# Autodesk Inventor assembly: base
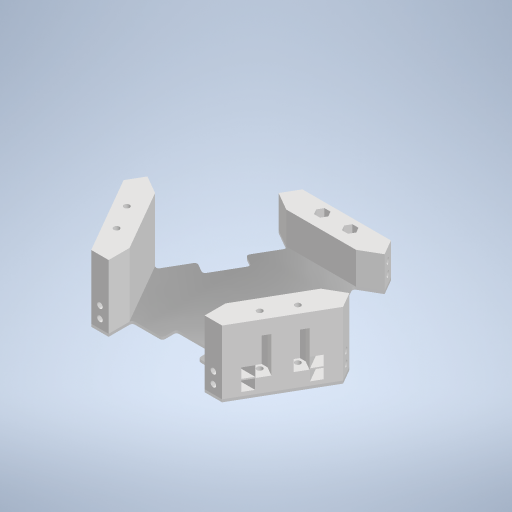
[picture p0: Inventor's stored thumbnail of the model, 512x512]
Saved by Autodesk Inventor 2024.1 (Build 281209000, 209)
## iProperties
Created: 2025-02-03
Part Number: base
Document SubType Name: Assembly
Designer: hibik
Author: hibik
## Documents named in this file (4)
- C:\Users\hibik\Documents\Robomech\RESCUE\ORCA\hard\flame_base\base.iam
- C:\Users\hibik\Documents\Robomech\RESCUE\ORCA\hard\flame_base\base_plate.ipt
- C:\Users\hibik\Documents\Robomech\RESCUE\ORCA\hard\flame_base\base_plate_towheel.ipt
- C:\Users\hibik\Documents\Robomech\RESCUE\ORCA\hard\flame_base\base_plate_towheel_front.ipt
## Components (4 placed, 3 different names)
1. base_plate:1 — メイト:3, フラッシュ:1, フラッシュ:6, 挿入:1, 挿入:2, 挿入:3, 挿入:4
2. base_plate_towheel:3 — メイト:3, フラッシュ:1, フラッシュ:6
3. base_plate_towheel_front:1 — 挿入:1, 挿入:2
4. base_plate_towheel_front:2 — 挿入:3, 挿入:4
## Relationships (7: Insert 4, Flush 2, Mate 1)
- メイト:3 [Mate]: base_plate:1 ↔ base_plate_towheel:3
- フラッシュ:1 [Flush]: base_plate:1 ↔ base_plate_towheel:3
- フラッシュ:6 [Flush]: base_plate:1 ↔ base_plate_towheel:3
- 挿入:1 [Insert]: base_plate:1 ↔ base_plate_towheel_front:1
- 挿入:2 [Insert]: base_plate:1 ↔ base_plate_towheel_front:1
- 挿入:3 [Insert]: base_plate:1 ↔ base_plate_towheel_front:2
- 挿入:4 [Insert]: base_plate:1 ↔ base_plate_towheel_front:2
